# Autodesk Inventor assembly: ASY mixer 2
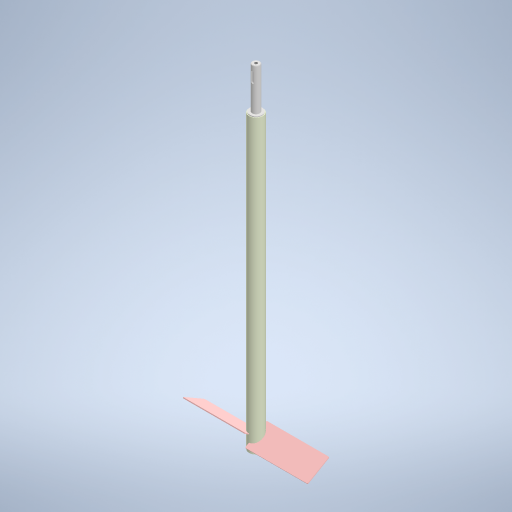
[picture p0: Inventor's stored thumbnail of the model, 512x512]
Saved by Autodesk Inventor 2023.2 (Build 272271030, 271C)
## iProperties
Created: 2023-08-07
Part Number: ASY mixer 2
Document SubType Name: Assembly
Designer: admin
Author: admin
## Documents named in this file (4)
- C:\Users\admin\My Drive (bigstupidbeast@gmail.com)\Inventor\StoTSy Furmanovo\CAD\Mixer 1\ASY mixer 2.iam
- C:\Users\admin\My Drive (bigstupidbeast@gmail.com)\Inventor\StoTSy Furmanovo\CAD\Mixer 1\shaft 3.ipt
- C:\Users\admin\My Drive (bigstupidbeast@gmail.com)\Inventor\StoTSy Furmanovo\CAD\Mixer 1\vane mixer.ipt
- C:\Users\admin\My Drive (bigstupidbeast@gmail.com)\Inventor\StoTSy Furmanovo\CAD\Mixer 1\shaft 2.ipt
## Components (4 placed, 3 different names)
1. shaft 3:1 — Rigid:1, Rigid:2, Rigid:3
2. vane mixer:1 — Flush:1, Rigid:1
3. vane mixer:2 — Rigid:2
4. shaft 2:1 — Rigid:3
## Relationships (4: WeldJoint 3, Flush 1)
- Flush:1: vane mixer:1
- Rigid:1 [WeldJoint] (-30 mm): shaft 3:1 ↔ vane mixer:1
- Rigid:2 [WeldJoint] (-30 mm): shaft 3:1 ↔ vane mixer:2
- Rigid:3 [WeldJoint] (-2 mm): shaft 3:1 ↔ shaft 2:1
